# Autodesk Inventor assembly: Scanning_setup_v1
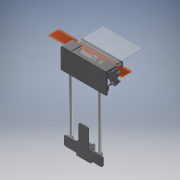
[picture p0: Inventor's stored thumbnail of the model, 180x180]
Saved by Autodesk Inventor 2019 (Build 230136000, 136)
## iProperties
Created: 2018-10-30
Part Number: Scanning_setup_v1
Document SubType Name: Assembly
Designer: Gianpietro
Author: Gianpietro
## Documents named in this file (11)
- C:\Giampo\Fotografia\Negative viewing & scanning\Scanning_setup_v1\scanning_setup_v1.1.iam
- C:\Giampo\Fotografia\Negative viewing & scanning\Scanning_setup_v1\camera_base_v1.1.ipt
- C:\Giampo\Fotografia\Negative viewing & scanning\Scanning_setup_v1\aluminium_bar_D8_L250.ipt
- C:\Giampo\Fotografia\Negative viewing & scanning\Scanning_setup_v1\film_holder_3_frames_v1.1_with_writing.ipt
- C:\Giampo\Fotografia\Negative viewing & scanning\Scanning_setup_v1\film_holder_3_frames_v1.1.ipt
- C:\Giampo\Fotografia\Negative viewing & scanning\Scanning_setup_v1\film_model_6_frames.ipt
- C:\Giampo\Fotografia\Negative viewing & scanning\Scanning_setup_v1\negative_holder_sleigh_v1.1.ipt
- C:\Users\Gianpietro\Documents\Inventor\Content Center Files\R2019\en-US\SS-ISO 1207\ISO 1207 - M4 x 25SS-ISO.ipt
- C:\Giampo\Fotografia\Negative viewing & scanning\Scanning_setup_v1\sleigh_base_v1.ipt
- C:\Users\Gianpietro\Documents\Inventor\Content Center Files\R2019\en-US\ISO 4032(2)\ISO 4032 - M4 - ISO.ipt
- C:\Giampo\Fotografia\Negative viewing & scanning\Scanning_setup_v1\polypropylene_sheet_120x120.ipt
## Components (27 placed, 10 different names)
1. camera_base_v1.1:1 — Cylindrical:1, Cylindrical:2, Flush:4, Flush:5, Angle:1, Angle:2
2. aluminium_bar_D8_L250:1 — Cylindrical:2, Flush:4, Angle:2, Cylindrical:9, Mate:17
3. aluminium_bar_D8_L250:2 — Cylindrical:1, Flush:5, Angle:1, Cylindrical:10
4. film_holder_3_frames_v1.1_with_writing:1 — Mate:5, Flush:1, Flush:2, Mate:7, Mate:8
5. film_holder_3_frames_v1.1:1 — Mate:3, Mate:4, Flush:1, Flush:2, Mate:6
6. film_model_6_frames:1 — Mate:3, Mate:4, Mate:5, Mate:6
7. negative_holder_sleigh_v1.1:1 — Mate:7, Mate:8, Cylindrical:3, Cylindrical:4, Cylindrical:5, Cylindrical:6, Cylindrical:7, Cylindrical:8, Mate:12, Mate:15, Angle:4, Mate:16, Mate:27, Mate:28, Angle:11, Angle:12, Mate:29, Mate:30, Mate:31, Mate:32, Mate:33, Angle:13, Angle:14, Angle:15, Angle:16, Mate:34, Mate:35, Angle:17, Mate:36, Mate:37, Mate:38
8. SS ISO 1207 M4 x 25:1 — Cylindrical:3, Mate:12, Cylindrical:18
9. SS ISO 1207 M4 x 25:2 — Cylindrical:4, Cylindrical:17, Mate:38
10. SS ISO 1207 M4 x 25:3 — Cylindrical:5, Cylindrical:19, Mate:37
11. SS ISO 1207 M4 x 25:4 — Cylindrical:6, Cylindrical:20, Mate:36
12. SS ISO 1207 M4 x 25:5 — Cylindrical:7, Cylindrical:22, Mate:34
13. SS ISO 1207 M4 x 25:6 — Cylindrical:8, Cylindrical:21, Mate:35, Angle:17
14. sleigh_base_v1:1 — Mate:15, Angle:4, Mate:16, Cylindrical:9, Cylindrical:10, Mate:17, Mate:18, Angle:5, Cylindrical:11, Cylindrical:12, Cylindrical:13, Cylindrical:14, Cylindrical:15, Cylindrical:16, Mate:19, Mate:20, Mate:21, Mate:22, Mate:23, Angle:6, Angle:7, Angle:8, Angle:9, Angle:10, Mate:24, Mate:25, Mate:26, Mate:27
15. ISO 4032 M4:1 — Mate:18, Angle:5, Cylindrical:11
16. ISO 4032 M4:2 — Cylindrical:12, Mate:21, Angle:7
17. ISO 4032 M4:3 — Cylindrical:13, Mate:23, Angle:6
18. ISO 4032 M4:4 — Cylindrical:15, Mate:22, Angle:10
19. ISO 4032 M4:5 — Cylindrical:16, Mate:19, Angle:9
20. ISO 4032 M4:6 — Cylindrical:14, Mate:20, Angle:8
21. polypropylene_sheet_120x120:1 — Mate:24, Mate:25, Mate:26
22. ISO 4032 M4:7 — Cylindrical:17, Mate:28, Angle:11
23. ISO 4032 M4:8 — Cylindrical:20, Mate:30, Angle:16
24. ISO 4032 M4:9 — Cylindrical:19, Mate:33, Angle:13
25. ISO 4032 M4:10 — Cylindrical:22, Mate:32, Angle:14
26. ISO 4032 M4:11 — Cylindrical:21, Mate:31, Angle:15
27. ISO 4032 M4:12 — Cylindrical:18, Angle:12, Mate:29
## Relationships (73: Mate 31, CylindricalJoint 22, Angle 16, Flush 4)
- Cylindrical:1: camera_base_v1.1:1 ↔ aluminium_bar_D8_L250:2
- Cylindrical:2: camera_base_v1.1:1 ↔ aluminium_bar_D8_L250:1
- Mate:3: film_holder_3_frames_v1.1:1 ↔ film_model_6_frames:1
- Mate:4 (1.5 mm): film_holder_3_frames_v1.1:1 ↔ film_model_6_frames:1
- Mate:5: film_holder_3_frames_v1.1_with_writing:1 ↔ film_model_6_frames:1
- Flush:1: film_holder_3_frames_v1.1_with_writing:1 ↔ film_holder_3_frames_v1.1:1
- Flush:2: film_holder_3_frames_v1.1_with_writing:1 ↔ film_holder_3_frames_v1.1:1
- Mate:6 (3.5 mm): film_holder_3_frames_v1.1:1 ↔ film_model_6_frames:1
- Flush:4: camera_base_v1.1:1 ↔ aluminium_bar_D8_L250:1
- Flush:5: camera_base_v1.1:1 ↔ aluminium_bar_D8_L250:2
- Mate:7 (0.2 mm): film_holder_3_frames_v1.1_with_writing:1 ↔ negative_holder_sleigh_v1.1:1
- Mate:8 (0.2 mm): film_holder_3_frames_v1.1_with_writing:1 ↔ negative_holder_sleigh_v1.1:1
- Cylindrical:3: negative_holder_sleigh_v1.1:1 ↔ SS ISO 1207 M4 x 25:1
- Cylindrical:4: negative_holder_sleigh_v1.1:1 ↔ SS ISO 1207 M4 x 25:2
- Cylindrical:5: negative_holder_sleigh_v1.1:1 ↔ SS ISO 1207 M4 x 25:3
- Cylindrical:6: negative_holder_sleigh_v1.1:1 ↔ SS ISO 1207 M4 x 25:4
- Cylindrical:7: negative_holder_sleigh_v1.1:1 ↔ SS ISO 1207 M4 x 25:5
- Cylindrical:8: negative_holder_sleigh_v1.1:1 ↔ SS ISO 1207 M4 x 25:6
- Mate:12: negative_holder_sleigh_v1.1:1 ↔ SS ISO 1207 M4 x 25:1
- Angle:1 (0 deg): camera_base_v1.1:1 ↔ aluminium_bar_D8_L250:2
- Angle:2 (0 deg): camera_base_v1.1:1 ↔ aluminium_bar_D8_L250:1
- Mate:15: negative_holder_sleigh_v1.1:1 ↔ sleigh_base_v1:1
- Angle:4 (180 deg): negative_holder_sleigh_v1.1:1 ↔ sleigh_base_v1:1
- Mate:16: negative_holder_sleigh_v1.1:1 ↔ sleigh_base_v1:1
- Cylindrical:9: aluminium_bar_D8_L250:1 ↔ sleigh_base_v1:1
- Cylindrical:10: aluminium_bar_D8_L250:2 ↔ sleigh_base_v1:1
- Mate:17: aluminium_bar_D8_L250:1 ↔ sleigh_base_v1:1
- Mate:18 (0.2 mm): sleigh_base_v1:1 ↔ ISO 4032 M4:1
- Angle:5 (0 deg): sleigh_base_v1:1 ↔ ISO 4032 M4:1
- Cylindrical:11: sleigh_base_v1:1 ↔ ISO 4032 M4:1
- Cylindrical:12: sleigh_base_v1:1 ↔ ISO 4032 M4:2
- Cylindrical:13: sleigh_base_v1:1 ↔ ISO 4032 M4:3
- Cylindrical:14: sleigh_base_v1:1 ↔ ISO 4032 M4:6
- Cylindrical:15: sleigh_base_v1:1 ↔ ISO 4032 M4:4
- Cylindrical:16: sleigh_base_v1:1 ↔ ISO 4032 M4:5
- Mate:19 (0.2 mm): sleigh_base_v1:1 ↔ ISO 4032 M4:5
- Mate:20 (0.2 mm): sleigh_base_v1:1 ↔ ISO 4032 M4:6
- Mate:21 (0.2 mm): sleigh_base_v1:1 ↔ ISO 4032 M4:2
- Mate:22 (0.2 mm): sleigh_base_v1:1 ↔ ISO 4032 M4:4
- Mate:23 (0.2 mm): sleigh_base_v1:1 ↔ ISO 4032 M4:3
- Angle:6 (0 deg): sleigh_base_v1:1 ↔ ISO 4032 M4:3
- Angle:7 (0 deg): sleigh_base_v1:1 ↔ ISO 4032 M4:2
- Angle:8 (0 deg): sleigh_base_v1:1 ↔ ISO 4032 M4:6
- Angle:9 (0 deg): sleigh_base_v1:1 ↔ ISO 4032 M4:5
- Angle:10 (0 deg): sleigh_base_v1:1 ↔ ISO 4032 M4:4
- Mate:24 (0.1 mm): sleigh_base_v1:1 ↔ polypropylene_sheet_120x120:1
- Mate:25: sleigh_base_v1:1 ↔ polypropylene_sheet_120x120:1
- Mate:26: sleigh_base_v1:1 ↔ polypropylene_sheet_120x120:1
- Mate:27 (30 mm): negative_holder_sleigh_v1.1:1 ↔ sleigh_base_v1:1
- Cylindrical:17: SS ISO 1207 M4 x 25:2 ↔ ISO 4032 M4:7
- Mate:28: negative_holder_sleigh_v1.1:1 ↔ ISO 4032 M4:7
- Angle:11 (0 deg): negative_holder_sleigh_v1.1:1 ↔ ISO 4032 M4:7
- Cylindrical:18: SS ISO 1207 M4 x 25:1 ↔ ISO 4032 M4:12
- Angle:12 (0 deg): negative_holder_sleigh_v1.1:1 ↔ ISO 4032 M4:12
- Mate:29: negative_holder_sleigh_v1.1:1 ↔ ISO 4032 M4:12
- Cylindrical:19: SS ISO 1207 M4 x 25:3 ↔ ISO 4032 M4:9
- Cylindrical:20: SS ISO 1207 M4 x 25:4 ↔ ISO 4032 M4:8
- Cylindrical:21: SS ISO 1207 M4 x 25:6 ↔ ISO 4032 M4:11
- Cylindrical:22: SS ISO 1207 M4 x 25:5 ↔ ISO 4032 M4:10
- Mate:30: negative_holder_sleigh_v1.1:1 ↔ ISO 4032 M4:8
- Mate:31: negative_holder_sleigh_v1.1:1 ↔ ISO 4032 M4:11
- Mate:32: negative_holder_sleigh_v1.1:1 ↔ ISO 4032 M4:10
- Mate:33: negative_holder_sleigh_v1.1:1 ↔ ISO 4032 M4:9
- Angle:13 (0 deg): negative_holder_sleigh_v1.1:1 ↔ ISO 4032 M4:9
- Angle:14 (0 deg): negative_holder_sleigh_v1.1:1 ↔ ISO 4032 M4:10
- Angle:15 (0 deg): negative_holder_sleigh_v1.1:1 ↔ ISO 4032 M4:11
- Angle:16 (0 deg): negative_holder_sleigh_v1.1:1 ↔ ISO 4032 M4:8
- Mate:34: negative_holder_sleigh_v1.1:1 ↔ SS ISO 1207 M4 x 25:5
- Mate:35: negative_holder_sleigh_v1.1:1 ↔ SS ISO 1207 M4 x 25:6
- Angle:17 (0 deg): negative_holder_sleigh_v1.1:1 ↔ SS ISO 1207 M4 x 25:6
- Mate:36: negative_holder_sleigh_v1.1:1 ↔ SS ISO 1207 M4 x 25:4
- Mate:37: negative_holder_sleigh_v1.1:1 ↔ SS ISO 1207 M4 x 25:3
- Mate:38: negative_holder_sleigh_v1.1:1 ↔ SS ISO 1207 M4 x 25:2
